# Autodesk Inventor assembly: Assembly1
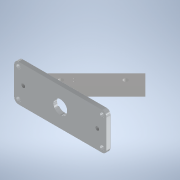
[picture p0: Inventor's stored thumbnail of the model, 180x180]
Saved by Autodesk Inventor 2022.2 (Build 262287010, 287A)
## iProperties
Created: 2022-05-04
Part Number: Assembly1
Document SubType Name: Assembly
Designer: Korch
Author: Korch
## Documents named in this file (3)
- C:\Users\Usuario\Desktop\Faculdade\modelagem_3D\motor_cilindro_unico\Assembly1.iam
- C:\Users\Usuario\Desktop\Faculdade\modelagem_3D\motor_cilindro_unico\base_plate.ipt
- C:\Users\Usuario\Desktop\Faculdade\modelagem_3D\motor_cilindro_unico\main_frame.ipt
## Components (2 placed, 2 different names)
1. base_plate:1 — Rigid:1
2. main_frame:1 — Rigid:1
## Relationships (1: WeldJoint 1)
- Rigid:1 [WeldJoint]: base_plate:1 ↔ main_frame:1
